# Autodesk Inventor assembly: Assembly_Autofocus_ke400_adjustable
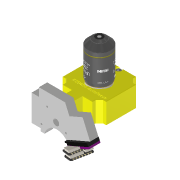
[picture p0: Inventor's stored thumbnail of the model, 180x180]
Saved by Autodesk Inventor 2022 (Build 260153000, 153)
## iProperties
Created: 2023-06-13
Part Number: Assembly_Autofocus_ke400_adjustable
Document SubType Name: Assembly
Designer: diederichbenedict
Author: diederichbenedict
## Documents named in this file (15)
- C:\Users\diederichbenedict\Dropbox\Dokumente\Promotion\PROJECTS\openUC2-CAD\INVENTOR\Assembly_Autofocus_ke400_adjustable.iam
- C:\Users\diederichbenedict\Dropbox\Dokumente\Promotion\PROJECTS\openUC2-CAD\INVENTOR\20_Cube_Insert_Autofocus_KES400a_mirrorinsert.ipt
- C:\Users\diederichbenedict\Dropbox\Dokumente\Promotion\PROJECTS\openUC2-CAD\INVENTOR\20_Cube_Insert_Autofocus_KES400a_mirrorinsert_mirrorholder.ipt
- C:\Users\diederichbenedict\Dropbox\Dokumente\Promotion\PROJECTS\openUC2-CAD\INVENTOR\20_Cube_Insert_Autofocus_KES400a_mirrorinsert_alignmenttube.ipt
- C:\Users\diederichbenedict\Dropbox\Dokumente\Promotion\PROJECTS\openUC2-CAD\INVENTOR\Assembly_Cube_SEEED_Xiao_Sense_Camera_adapter_v3.iam
- C:\Users\diederichbenedict\Dropbox\Dokumente\Promotion\PROJECTS\openUC2-CAD\INVENTOR\00_KES400.iam
- C:\Users\diederichbenedict\Dropbox\Dokumente\Promotion\PROJECTS\openUC2-CAD\INVENTOR\00_Xia_KES400_Lens_adapter.ipt
- C:\Users\diederichbenedict\Dropbox\Dokumente\Promotion\PROJECTS\openUC2-CAD\INVENTOR\00_KES400A_base.ipt
- C:\Users\diederichbenedict\Dropbox\Dokumente\Promotion\PROJECTS\openUC2-CAD\INVENTOR\Camera_Autofocus_Mount.iam
- C:\Users\diederichbenedict\Dropbox\Dokumente\Promotion\PROJECTS\openUC2-CAD\INVENTOR\Jordiscope_XYZ_Case_Printed\00_M3_Ballheaded_screw_20mm.ipt
- C:\Users\diederichbenedict\Documents\Inventor\Content Center Files\R2022\de-DE\DIN 912\DIN 912 - M2 x 0.4 x 20 x 19.ipt
- C:\Users\diederichbenedict\Dropbox\Dokumente\Promotion\PROJECTS\openUC2-CAD\INVENTOR\Jordiscope_XYZ_Case_Printed\00_Spring_3mm_3mm.ipt
- C:\Users\diederichbenedict\Dropbox\Dokumente\Promotion\PROJECTS\openUC2-CAD\INVENTOR\00_Microscope_objective_10x.ipt
- C:\Users\diederichbenedict\Dropbox\Dokumente\Promotion\PROJECTS\openUC2-CAD\INVENTOR\content\DIN 912\DIN 912 - M3 x 0,5 x 10 x 8,75.ipt
- C:\Users\diederichbenedict\Dropbox\Dokumente\Promotion\PROJECTS\openUC2-CAD\INVENTOR\content\DIN 912\DIN 912 - M3 x 0,5 x 16 x 20.ipt
## Components (21 placed, 14 different names)
1. 20_Cube_Insert_Autofocus_KES400a_mirrorinsert:1 — Fluchtend:1, Fluchtend:2, Fluchtend:3, Fluchtend:4, Einfügen:2, Winkel:2, Einfügen:4, Einfügen:5, Einfügen:6, Einfügen:10, Einfügen:11, Passend:1, Einfügen:12, Einfügen:13, Passend:2, Einfügen:14, Einfügen:15
2. 20_Cube_Insert_Autofocus_KES400a_mirrorinsert_mirrorholder:1 — Fluchtend:1, Fluchtend:2, Einfügen:8, Einfügen:9
3. 20_Cube_Insert_Autofocus_KES400a_mirrorinsert_alignmenttube:1 — Fluchtend:3, Fluchtend:4
4. Assembly_Cube_SEEED_Xiao_Sense_Camera_adapter_v3:1 [sub-assembly] — Einfügen:1, Winkel:1, Fluchtend:5, Fluchtend:6
5. 00_KES400:1 [sub-assembly] — Einfügen:1, Winkel:1, Einfügen:3
6. 00_Xia_KES400_Lens_adapter:1 — Fluchtend:5, Fluchtend:6
7. 00_KES400A_base:1 — Einfügen:2, Winkel:2, Einfügen:3, Einfügen:7, Winkel:3
8. Camera_Autofocus_Mount:1 [sub-assembly] — Einfügen:7, Winkel:3
9. 00_M3_Ballheaded_screw_20mm:1 — Einfügen:4
10. 00_M3_Ballheaded_screw_20mm:2 — Einfügen:5
11. 00_M3_Ballheaded_screw_20mm:3 — Einfügen:6
12. DIN 912 - ersetzt durch DIN EN ISO 4762 M2 x 20:1 — Einfügen:8
13. DIN 912 - ersetzt durch DIN EN ISO 4762 M2 x 20:2 — Einfügen:9
14. 00_Spring_3mm_3mm:1 — Einfügen:10
15. 00_Spring_3mm_3mm:2 — Einfügen:11
16. 00_Microscope_objective_10x:1 — Passend:1
17. DIN 912 - ersetzt durch DIN EN ISO 4762 M3 x 10:1 — Einfügen:12
18. DIN 912 - ersetzt durch DIN EN ISO 4762 M3 x 10:2 — Einfügen:13
19. DIN 912 - ersetzt durch DIN EN ISO 4762 M3 x 10:3 — Passend:2
20. DIN 912 - ersetzt durch DIN EN ISO 4762 M3 x 16:1 — Einfügen:14
21. DIN 912 - ersetzt durch DIN EN ISO 4762 M3 x 16:2 — Einfügen:15
## Relationships (26: Insert 15, Flush 6, Angle 3, Mate 2)
- Fluchtend:1 [Flush]: 20_Cube_Insert_Autofocus_KES400a_mirrorinsert:1 ↔ 20_Cube_Insert_Autofocus_KES400a_mirrorinsert_mirrorholder:1
- Fluchtend:2 [Flush]: 20_Cube_Insert_Autofocus_KES400a_mirrorinsert:1 ↔ 20_Cube_Insert_Autofocus_KES400a_mirrorinsert_mirrorholder:1
- Fluchtend:3 [Flush]: 20_Cube_Insert_Autofocus_KES400a_mirrorinsert:1 ↔ 20_Cube_Insert_Autofocus_KES400a_mirrorinsert_alignmenttube:1
- Fluchtend:4 [Flush]: 20_Cube_Insert_Autofocus_KES400a_mirrorinsert:1 ↔ 20_Cube_Insert_Autofocus_KES400a_mirrorinsert_alignmenttube:1
- Einfügen:1 [Insert] (10 mm): Assembly_Cube_SEEED_Xiao_Sense_Camera_adapter_v3:1 ↔ 00_KES400:1
- Winkel:1 [Angle] (0 deg): Assembly_Cube_SEEED_Xiao_Sense_Camera_adapter_v3:1 ↔ 00_KES400:1
- Fluchtend:5 [Flush]: Assembly_Cube_SEEED_Xiao_Sense_Camera_adapter_v3:1 ↔ 00_Xia_KES400_Lens_adapter:1
- Fluchtend:6 [Flush]: Assembly_Cube_SEEED_Xiao_Sense_Camera_adapter_v3:1 ↔ 00_Xia_KES400_Lens_adapter:1
- Einfügen:2 [Insert]: 20_Cube_Insert_Autofocus_KES400a_mirrorinsert:1 ↔ 00_KES400A_base:1
- Winkel:2 [Angle] (0 deg): 20_Cube_Insert_Autofocus_KES400a_mirrorinsert:1 ↔ 00_KES400A_base:1
- Einfügen:3 [Insert] (10 mm): 00_KES400:1 ↔ 00_KES400A_base:1
- Einfügen:4 [Insert] (-5 mm): 20_Cube_Insert_Autofocus_KES400a_mirrorinsert:1 ↔ 00_M3_Ballheaded_screw_20mm:1
- Einfügen:5 [Insert] (-5 mm): 20_Cube_Insert_Autofocus_KES400a_mirrorinsert:1 ↔ 00_M3_Ballheaded_screw_20mm:2
- Einfügen:6 [Insert] (-5 mm): 20_Cube_Insert_Autofocus_KES400a_mirrorinsert:1 ↔ 00_M3_Ballheaded_screw_20mm:3
- Einfügen:7 [Insert]: 00_KES400A_base:1 ↔ Camera_Autofocus_Mount:1
- Winkel:3 [Angle] (0 deg): 00_KES400A_base:1 ↔ Camera_Autofocus_Mount:1
- Einfügen:8 [Insert]: 20_Cube_Insert_Autofocus_KES400a_mirrorinsert_mirrorholder:1 ↔ DIN 912 - ersetzt durch DIN EN ISO 4762 M2 x 20:1
- Einfügen:9 [Insert]: 20_Cube_Insert_Autofocus_KES400a_mirrorinsert_mirrorholder:1 ↔ DIN 912 - ersetzt durch DIN EN ISO 4762 M2 x 20:2
- Einfügen:10 [Insert] (-5 mm): 20_Cube_Insert_Autofocus_KES400a_mirrorinsert:1 ↔ 00_Spring_3mm_3mm:1
- Einfügen:11 [Insert] (-5 mm): 20_Cube_Insert_Autofocus_KES400a_mirrorinsert:1 ↔ 00_Spring_3mm_3mm:2
- Passend:1 [Mate]: 20_Cube_Insert_Autofocus_KES400a_mirrorinsert:1 ↔ 00_Microscope_objective_10x:1
- Einfügen:12 [Insert]: 20_Cube_Insert_Autofocus_KES400a_mirrorinsert:1 ↔ DIN 912 - ersetzt durch DIN EN ISO 4762 M3 x 10:1
- Einfügen:13 [Insert]: 20_Cube_Insert_Autofocus_KES400a_mirrorinsert:1 ↔ DIN 912 - ersetzt durch DIN EN ISO 4762 M3 x 10:2
- Passend:2 [Mate]: 20_Cube_Insert_Autofocus_KES400a_mirrorinsert:1 ↔ DIN 912 - ersetzt durch DIN EN ISO 4762 M3 x 10:3
- Einfügen:14 [Insert]: 20_Cube_Insert_Autofocus_KES400a_mirrorinsert:1 ↔ DIN 912 - ersetzt durch DIN EN ISO 4762 M3 x 16:1
- Einfügen:15 [Insert]: 20_Cube_Insert_Autofocus_KES400a_mirrorinsert:1 ↔ DIN 912 - ersetzt durch DIN EN ISO 4762 M3 x 16:2
